# Autodesk Inventor assembly: ControlHousing
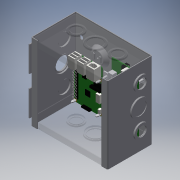
[picture p0: Inventor's stored thumbnail of the model, 180x180]
Saved by Autodesk Inventor 2016 (Build 200138000, 138)
## iProperties
Company: Unknown
Created: 2016-08-11
Part Number: ControlHousing
Description: Unknown
Document SubType Name: Assembly
Designer: jfixelle
Sending System: Unknown
Preprocessor: PSStep 14.0
Title: S:/STOCK/7-COMMERCIAL/CHKO/chko663.stp
Author: Unknown
Revision Number: NONE
## Documents named in this file (26)
- E:\jfixelle\Documents\APC\GitRepo\Control\IAM\ControlHousing.iam
- E:\jfixelle\Downloads\loc13368.ipt
- E:\jfixelle\Downloads\COM55083-4.ipt
- E:\jfixelle\Downloads\COM55563-4.ipt
- E:\jfixelle\Downloads\COM55989.ipt
- E:\jfixelle\Downloads\HNG11000.iam
- E:\jfixelle\Documents\APC\GitRepo\Control\IAM\PiB+.ipt
- E:\jfixelle\Documents\APC\GitRepo\Control\IAM\ControlBoard_New.ipt
- E:\jfixelle\Documents\APC\GitRepo\PCB_Libs\3DParts\IDC_10Pos.ipt
- E:\jfixelle\Documents\APC\GitRepo\PCB_Libs\3DParts\IDC_16Pos.ipt
- E:\jfixelle\Documents\APC\GitRepo\PCB_Libs\3DParts\Molex_MiniFitJR_4Pos.ipt
- E:\jfixelle\Documents\APC\GitRepo\PCB_Libs\3DParts\RJE051AA1310.ipt
- E:\jfixelle\Documents\APC\GitRepo\PCB_Libs\3DParts\H11L1M.ipt
- E:\jfixelle\Documents\APC\GitRepo\PCB_Libs\3DParts\Screw_Terminal_3Pos.ipt
- E:\jfixelle\Documents\APC\GitRepo\PCB_Libs\3DParts\Keystone1056_12_5mmCoinCell.ipt
- E:\jfixelle\Documents\APC\GitRepo\PCB_Libs\3DParts\Inductor_SMD_12mm.ipt
- E:\jfixelle\Documents\APC\GitRepo\PCB_Libs\3DParts\SMTElectro4x4x6_5.ipt
- E:\jfixelle\Documents\APC\GitRepo\PCB_Libs\3DParts\CFS-20632768EZBB_Watch_Crystal.ipt
- E:\jfixelle\Documents\APC\GitRepo\PCB_Libs\3DParts\BK-6013_MiniATC_Fuse_Holder.ipt
- E:\jfixelle\Documents\APC\GitRepo\PCB_Libs\3DParts\Mini-ATC_FUse.ipt
- E:\jfixelle\Documents\APC\GitRepo\PCB_Libs\3DParts\16mm_7_2mmDiskPTC.ipt
- E:\jfixelle\Documents\APC\GitRepo\PCB_Libs\3DParts\9mm_5mm_MOV.ipt
- E:\jfixelle\Documents\APC\GitRepo\PCB_Libs\3DParts\PIC16LF1946.ipt
- E:\jfixelle\Documents\APC\GitRepo\PCB_Libs\3DParts\HC49_XTAL.ipt
- E:\jfixelle\Documents\APC\GitRepo\PCB_Libs\3DParts\11mm_Board_Support.ipt
- E:\jfixelle\Documents\APC\GitRepo\Control\IAM\ControlHousing\AIP\Cable and Harness\ControlHousing.Harness1.iam
## Components (38 placed, 27 different names)
1. NAUO4
2. NAUO5
3. NAUO6
4. NAUO7 — Mate:56, Angle:8, Mate:68, Angle:13
5. NAUO8
6. NAUO9 [sub-assembly]
7. NAUO10 [sub-assembly]
8. PiB+:1 — Mate:60, Mate:61, Mate:62, Mate:63, Mate:64, Mate:65, Mate:66, Mate:67, Angle:9, Angle:10, Angle:11, Angle:12, Angle:13
9. ControlBoard_New:1 — Mate:2, Mate:3, Mate:4, Mate:5, Mate:6, Mate:7, Mate:8, Mate:9, Mate:10, Mate:11, Mate:12, Mate:13, Mate:14, Mate:15, Flush:1, Flush:2, Mate:18, Mate:21, Mate:22, Mate:23, Mate:24, Angle:1, Mate:25, Mate:26, Flush:4, Flush:5, Flush:6, Mate:28, Mate:29, Flush:7, Mate:33, Mate:34, Mate:35, Mate:36, Mate:37, Mate:38, Mate:42, Mate:43, Angle:2, Mate:44, Mate:45, Angle:3, Mate:46, Flush:8, Flush:9, Mate:47, Flush:10, Flush:11, Mate:48, Mate:49, Mate:50, Mate:51, Mate:52, Mate:53, Mate:54, Mate:55, Angle:4, Angle:5, Angle:6, Angle:7, Angle:8, Mate:57, Mate:58, Mate:59
10. IDC_10Pos:1 — Mate:2, Mate:7, Mate:8
11. IDC_16Pos:1 — Mate:3, Mate:9, Mate:10
12. Molex_MiniFitJR_4Pos:1 — Mate:4, Mate:5, Mate:6
13. RJE051AA1310:1 — Mate:11, Mate:12, Mate:13, Mate:16
14. H11L1M:1 — Mate:14, Flush:2, Flush:3
15. H11L1M:2 — Mate:15, Flush:1, Mate:16, Flush:3
16. Screw_Terminal_3Pos:1 — Mate:18, Mate:21, Mate:22
17. Keystone1056_12_5mmCoinCell:1 — Mate:23, Mate:24, Angle:1, Mate:27
18. Inductor_SMD_12mm:1 — Mate:25, Flush:4, Flush:5, Mate:30, Mate:31
19. Inductor_SMD_12mm:2 — Mate:26, Flush:6, Mate:27, Mate:32
20. SMTElectro4x4x6_5:1 — Mate:29, Mate:32, Flush:7
21. SMTElectro4x4x6_5:2 — Mate:28, Mate:30, Mate:31
22. CFS-20632768EZBB_Watch_Crystal:1 — Mate:33, Mate:34, Mate:35
23. BK-6013_MiniATC_Fuse_Holder:1 — Mate:36, Mate:37, Mate:38, Mate:39, Mate:40, Mate:41
24. Mini-ATC_FUse:1 — Mate:39, Mate:40, Mate:41
25. 16mm_7_2mmDiskPTC:1 — Mate:42, Mate:43, Angle:2
26. 9mm_5mm_MOV:1 — Mate:44, Mate:45, Angle:3
27. PIC16LF1946:1 — Mate:46, Flush:8, Flush:9
28. HC49_XTAL:1 — Mate:47, Flush:10, Flush:11
29. 11mm_Board_Support:1 — Mate:48, Mate:55, Angle:4
30. 11mm_Board_Support:2 — Mate:49, Mate:53, Angle:6, Mate:56
31. 11mm_Board_Support:3 — Mate:51, Mate:54, Angle:7
32. 11mm_Board_Support:4 — Mate:50, Mate:52, Angle:5
33. Screw_Terminal_3Pos:2 — Mate:57, Mate:58, Mate:59
34. 11mm_Board_Support:5 — Mate:60, Mate:66, Angle:9
35. 11mm_Board_Support:6 — Mate:61, Mate:65, Angle:11
36. 11mm_Board_Support:7 — Mate:63, Mate:64, Angle:12, Mate:68
37. 11mm_Board_Support:8 — Mate:62, Mate:67, Angle:10
38. Harness1 [sub-assembly]
## Relationships (88: Mate 64, Angle 13, Flush 11)
- Mate:2: ControlBoard_New:1 ↔ IDC_10Pos:1
- Mate:3: ControlBoard_New:1 ↔ IDC_16Pos:1
- Mate:4: ControlBoard_New:1 ↔ Molex_MiniFitJR_4Pos:1
- Mate:5: ControlBoard_New:1 ↔ Molex_MiniFitJR_4Pos:1
- Mate:6: ControlBoard_New:1 ↔ Molex_MiniFitJR_4Pos:1
- Mate:7: ControlBoard_New:1 ↔ IDC_10Pos:1
- Mate:8: ControlBoard_New:1 ↔ IDC_10Pos:1
- Mate:9: ControlBoard_New:1 ↔ IDC_16Pos:1
- Mate:10: ControlBoard_New:1 ↔ IDC_16Pos:1
- Mate:11: ControlBoard_New:1 ↔ RJE051AA1310:1
- Mate:12: ControlBoard_New:1 ↔ RJE051AA1310:1
- Mate:13: ControlBoard_New:1 ↔ RJE051AA1310:1
- Mate:14: ControlBoard_New:1 ↔ H11L1M:1
- Mate:15: ControlBoard_New:1 ↔ H11L1M:2
- Flush:1: ControlBoard_New:1 ↔ H11L1M:2
- Mate:16: RJE051AA1310:1 ↔ H11L1M:2
- Flush:2: ControlBoard_New:1 ↔ H11L1M:1
- Flush:3: H11L1M:1 ↔ H11L1M:2
- Mate:18: ControlBoard_New:1 ↔ Screw_Terminal_3Pos:1
- Mate:21: ControlBoard_New:1 ↔ Screw_Terminal_3Pos:1
- Mate:22: ControlBoard_New:1 ↔ Screw_Terminal_3Pos:1
- Mate:23: ControlBoard_New:1 ↔ Keystone1056_12_5mmCoinCell:1
- Mate:24: ControlBoard_New:1 ↔ Keystone1056_12_5mmCoinCell:1
- Angle:1 (0 deg): ControlBoard_New:1 ↔ Keystone1056_12_5mmCoinCell:1
- Mate:25: ControlBoard_New:1 ↔ Inductor_SMD_12mm:1
- Mate:26: ControlBoard_New:1 ↔ Inductor_SMD_12mm:2
- Flush:4 (6.35 mm): ControlBoard_New:1 ↔ Inductor_SMD_12mm:1
- Flush:5 (6.35 mm): ControlBoard_New:1 ↔ Inductor_SMD_12mm:1
- Flush:6 (6.35 mm): ControlBoard_New:1 ↔ Inductor_SMD_12mm:2
- Mate:27 (6.35 mm): Keystone1056_12_5mmCoinCell:1 ↔ Inductor_SMD_12mm:2
- Mate:28: ControlBoard_New:1 ↔ SMTElectro4x4x6_5:2
- Mate:29: ControlBoard_New:1 ↔ SMTElectro4x4x6_5:1
- Mate:30: Inductor_SMD_12mm:1 ↔ SMTElectro4x4x6_5:2
- Mate:31: Inductor_SMD_12mm:1 ↔ SMTElectro4x4x6_5:2
- Mate:32: Inductor_SMD_12mm:2 ↔ SMTElectro4x4x6_5:1
- Flush:7 (25.4 mm): ControlBoard_New:1 ↔ SMTElectro4x4x6_5:1
- Mate:33: ControlBoard_New:1 ↔ CFS-20632768EZBB_Watch_Crystal:1
- Mate:34: ControlBoard_New:1 ↔ CFS-20632768EZBB_Watch_Crystal:1
- Mate:35: ControlBoard_New:1 ↔ CFS-20632768EZBB_Watch_Crystal:1
- Mate:36: ControlBoard_New:1 ↔ BK-6013_MiniATC_Fuse_Holder:1
- Mate:37: ControlBoard_New:1 ↔ BK-6013_MiniATC_Fuse_Holder:1
- Mate:38: ControlBoard_New:1 ↔ BK-6013_MiniATC_Fuse_Holder:1
- Mate:39: BK-6013_MiniATC_Fuse_Holder:1 ↔ Mini-ATC_FUse:1
- Mate:40: BK-6013_MiniATC_Fuse_Holder:1 ↔ Mini-ATC_FUse:1
- Mate:41: BK-6013_MiniATC_Fuse_Holder:1 ↔ Mini-ATC_FUse:1
- Mate:42: ControlBoard_New:1 ↔ 16mm_7_2mmDiskPTC:1
- Mate:43: ControlBoard_New:1 ↔ 16mm_7_2mmDiskPTC:1
- Angle:2 (0 deg): ControlBoard_New:1 ↔ 16mm_7_2mmDiskPTC:1
- Mate:44: ControlBoard_New:1 ↔ 9mm_5mm_MOV:1
- Mate:45: ControlBoard_New:1 ↔ 9mm_5mm_MOV:1
- Angle:3 (0 deg): ControlBoard_New:1 ↔ 9mm_5mm_MOV:1
- Mate:46: ControlBoard_New:1 ↔ PIC16LF1946:1
- Flush:8 (24.4 mm): ControlBoard_New:1 ↔ PIC16LF1946:1
- Flush:9 (15 mm): ControlBoard_New:1 ↔ PIC16LF1946:1
- Mate:47: ControlBoard_New:1 ↔ HC49_XTAL:1
- Flush:10 (39.4 mm): ControlBoard_New:1 ↔ HC49_XTAL:1
- Flush:11 (27 mm): ControlBoard_New:1 ↔ HC49_XTAL:1
- Mate:48: ControlBoard_New:1 ↔ 11mm_Board_Support:1
- Mate:49: ControlBoard_New:1 ↔ 11mm_Board_Support:2
- Mate:50: ControlBoard_New:1 ↔ 11mm_Board_Support:4
- Mate:51: ControlBoard_New:1 ↔ 11mm_Board_Support:3
- Mate:52: ControlBoard_New:1 ↔ 11mm_Board_Support:4
- Mate:53: ControlBoard_New:1 ↔ 11mm_Board_Support:2
- Mate:54: ControlBoard_New:1 ↔ 11mm_Board_Support:3
- Mate:55: ControlBoard_New:1 ↔ 11mm_Board_Support:1
- Angle:4 (0 deg): ControlBoard_New:1 ↔ 11mm_Board_Support:1
- Angle:5 (0 deg): ControlBoard_New:1 ↔ 11mm_Board_Support:4
- Angle:6 (0 deg): ControlBoard_New:1 ↔ 11mm_Board_Support:2
- Angle:7 (0 deg): ControlBoard_New:1 ↔ 11mm_Board_Support:3
- Mate:56: NAUO7 ↔ 11mm_Board_Support:2
- Angle:8 (0 deg): NAUO7 ↔ ControlBoard_New:1
- Mate:57: ControlBoard_New:1 ↔ Screw_Terminal_3Pos:2
- Mate:58: ControlBoard_New:1 ↔ Screw_Terminal_3Pos:2
- Mate:59: ControlBoard_New:1 ↔ Screw_Terminal_3Pos:2
- Mate:60: PiB+:1 ↔ 11mm_Board_Support:5
- Mate:61: PiB+:1 ↔ 11mm_Board_Support:6
- Mate:62: PiB+:1 ↔ 11mm_Board_Support:8
- Mate:63: PiB+:1 ↔ 11mm_Board_Support:7
- Mate:64: PiB+:1 ↔ 11mm_Board_Support:7
- Mate:65: PiB+:1 ↔ 11mm_Board_Support:6
- Mate:66: PiB+:1 ↔ 11mm_Board_Support:5
- Mate:67: PiB+:1 ↔ 11mm_Board_Support:8
- Angle:9 (0 deg): PiB+:1 ↔ 11mm_Board_Support:5
- Angle:10 (0 deg): PiB+:1 ↔ 11mm_Board_Support:8
- Angle:11 (0 deg): PiB+:1 ↔ 11mm_Board_Support:6
- Angle:12 (0 deg): PiB+:1 ↔ 11mm_Board_Support:7
- Mate:68: NAUO7 ↔ 11mm_Board_Support:7
- Angle:13 (0 deg): NAUO7 ↔ PiB+:1
